# Autodesk Inventor assembly: Shifter Assembly
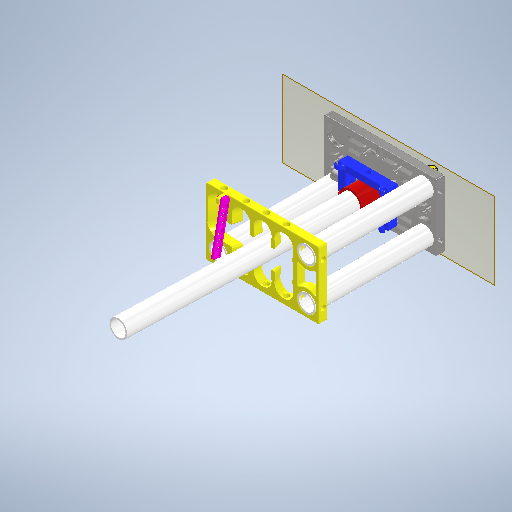
[picture p0: Inventor's stored thumbnail of the model, 512x512]
Saved by Autodesk Inventor 2025.2 (Build 292293000, 293)
## iProperties
Created: 2025-02-09
Part Number: Shifter Assembly
Document SubType Name: Assembly
Designer: eason
Author: eason
## Documents named in this file (8)
- C:\Users\eason\Desktop\Code\Unojoy-Simulator-Rig\CAD\Shifter\Shifter Assembly.iam
- C:\Users\eason\Desktop\Code\Unojoy-Simulator-Rig\CAD\Shifter\Shifter Joint 2.ipt
- C:\Users\eason\Desktop\Code\Unojoy-Simulator-Rig\CAD\Shifter\Shifter Joint.ipt
- C:\Users\eason\Desktop\Code\Unojoy-Simulator-Rig\CAD\Shifter\Shifter Support.ipt
- C:\Users\eason\Desktop\Code\Unojoy-Simulator-Rig\CAD\Shifter\Shifter Post.ipt
- C:\Users\eason\Desktop\Code\Unojoy-Simulator-Rig\CAD\Shifter\Shifter Gater.ipt
- C:\Users\eason\Desktop\Code\Unojoy-Simulator-Rig\CAD\Shifter\Reverse Lockout.ipt
- C:\Users\eason\Desktop\Code\Unojoy-Simulator-Rig\CAD\Shifter\Shifter PVC.ipt
## Components (9 placed, 7 different names)
1. Shifter Support:1 — Mate:10, Cylindrical:1, Cylindrical:2, Cylindrical:3, Mate:11, Mate:12, Mate:13, Insert:1
2. Shifter Post:1 — Cylindrical:1, Mate:11, Cylindrical:5, Mate:15
3. Shifter Post:2 — Cylindrical:2, Mate:12
4. Shifter Post:3 — Cylindrical:3, Mate:13
5. Shifter Joint 2:1 — Cylindrical:4, Tangent:1, Insert:1
6. Shifter Joint:1 — Cylindrical:4, Tangent:1, Cylindrical:6, Mate:16
7. Shifter Gater:1 — Cylindrical:5, Mate:15, Insert:2
8. Reverse Lockout:1 — Insert:2
9. Shifter PVC:1 — Cylindrical:6, Mate:16
## Relationships (15: Mate 6, CylindricalJoint 6, Insert 2, Tangent 1)
- Mate:10: Shifter Support:1
- Cylindrical:1: Shifter Support:1 ↔ Shifter Post:1
- Cylindrical:2: Shifter Support:1 ↔ Shifter Post:2
- Cylindrical:3: Shifter Support:1 ↔ Shifter Post:3
- Mate:11: Shifter Support:1 ↔ Shifter Post:1
- Mate:12: Shifter Support:1 ↔ Shifter Post:2
- Mate:13: Shifter Support:1 ↔ Shifter Post:3
- Cylindrical:4: Shifter Joint 2:1 ↔ Shifter Joint:1
- Tangent:1: Shifter Joint 2:1 ↔ Shifter Joint:1
- Cylindrical:5: Shifter Post:1 ↔ Shifter Gater:1
- Mate:15: Shifter Post:1 ↔ Shifter Gater:1
- Insert:1: Shifter Support:1 ↔ Shifter Joint 2:1
- Cylindrical:6: Shifter Joint:1 ↔ Shifter PVC:1
- Mate:16: Shifter Joint:1 ↔ Shifter PVC:1
- Insert:2: Shifter Gater:1 ↔ Reverse Lockout:1
